# Autodesk Inventor assembly: Assembly1
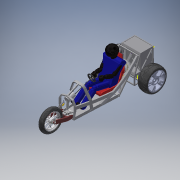
[picture p0: Inventor's stored thumbnail of the model, 180x180]
Saved by Autodesk Inventor 2019 (Build 230136000, 136)
## iProperties
Created: 2020-10-01
Part Number: Assembly1
Document SubType Name: Assembly
Designer: nabee
Author: nabee
## Documents named in this file (6)
- D:\Uni y2\Sem2\236\Design Project\Assembly1.iam
- D:\Uni y2\Sem2\236\Design Project\given cad\Design Project_Inventor CAD Files (1)\CARMODEL\Urban Transport Design Project_Master.iam
- D:\Uni y2\Sem2\236\Design Project\Cad files\My files\New motorhousing - Copy.ipt
- D:\Uni y2\Sem2\236\Design Project\Cad files\My files\gearbox.ipt
- D:\Uni y2\Sem2\236\Design Project\shock absorber.ipt
- D:\Uni y2\Sem2\236\Design Project\Cad files\My files\Updated Motor.ipt
## Components (6 placed, 5 different names)
1. Urban Transport Design Project_Master:1 [sub-assembly]
2. New motorhousing - Copy:2 — Mate:2, Mate:3, Mate:4, Mate:5, Flush:1, Mate:6, Flush:2, Mate:7, Mate:8, Mate:9
3. shock absorber:1 — Mate:6, Flush:2
4. gearbox:1 — Mate:2, Mate:3, Mate:4
5. Updated Motor:1 — Mate:7, Mate:8, Mate:9
6. shock absorber:2 — Mate:5, Flush:1
## Relationships (10: Mate 8, Flush 2)
- Mate:2: New motorhousing - Copy:2 ↔ gearbox:1
- Mate:3: New motorhousing - Copy:2 ↔ gearbox:1
- Mate:4: New motorhousing - Copy:2 ↔ gearbox:1
- Mate:5: New motorhousing - Copy:2 ↔ shock absorber:2
- Flush:1: New motorhousing - Copy:2 ↔ shock absorber:2
- Mate:6: New motorhousing - Copy:2 ↔ shock absorber:1
- Flush:2: New motorhousing - Copy:2 ↔ shock absorber:1
- Mate:7: New motorhousing - Copy:2 ↔ Updated Motor:1
- Mate:8 (5 mm): New motorhousing - Copy:2 ↔ Updated Motor:1
- Mate:9 (5 mm): New motorhousing - Copy:2 ↔ Updated Motor:1
